# Autodesk Inventor assembly: COMPONENTS
(part 4 of 4)
- C:\Users\rtreacy\Documents\Inventor\SNAP Enclosure 8x10x1.75 Ver1.A\drawings\SNAP Ver2 pack-n-go\Workgroups\NotInProject\RESC3216X70N_R460.ipt
- C:\Users\rtreacy\Documents\Inventor\SNAP Enclosure 8x10x1.75 Ver1.A\drawings\SNAP Ver2 pack-n-go\Workgroups\NotInProject\RESC3216X70N_R165.ipt
- C:\Users\rtreacy\Documents\Inventor\SNAP Enclosure 8x10x1.75 Ver1.A\drawings\SNAP Ver2 pack-n-go\Workgroups\NotInProject\RESC3216X70N_R74.ipt
- C:\Users\rtreacy\Documents\Inventor\SNAP Enclosure 8x10x1.75 Ver1.A\drawings\SNAP Ver2 pack-n-go\Workgroups\NotInProject\RESC3216X70N_R474.ipt
- C:\Users\rtreacy\Documents\Inventor\SNAP Enclosure 8x10x1.75 Ver1.A\drawings\SNAP Ver2 pack-n-go\Workgroups\NotInProject\TP107_GNDTP6.ipt
- C:\Users\rtreacy\Documents\Inventor\SNAP Enclosure 8x10x1.75 Ver1.A\drawings\SNAP Ver2 pack-n-go\Workgroups\NotInProject\TP107_GNDTP5.ipt
- C:\Users\rtreacy\Documents\Inventor\SNAP Enclosure 8x10x1.75 Ver1.A\drawings\SNAP Ver2 pack-n-go\Workgroups\NotInProject\TP107_GNDTP4.ipt
- C:\Users\rtreacy\Documents\Inventor\SNAP Enclosure 8x10x1.75 Ver1.A\drawings\SNAP Ver2 pack-n-go\Workgroups\NotInProject\TP107_GNDTP3.ipt
- C:\Users\rtreacy\Documents\Inventor\SNAP Enclosure 8x10x1.75 Ver1.A\drawings\SNAP Ver2 pack-n-go\Workgroups\NotInProject\TP107_GNDTP2.ipt
- C:\Users\rtreacy\Documents\Inventor\SNAP Enclosure 8x10x1.75 Ver1.A\drawings\SNAP Ver2 pack-n-go\Workgroups\NotInProject\TP107_GNDTP1.ipt
- C:\Users\rtreacy\Documents\Inventor\SNAP Enclosure 8x10x1.75 Ver1.A\drawings\SNAP Ver2 pack-n-go\Workgroups\NotInProject\TP107_TP1.ipt
- C:\Users\rtreacy\Documents\Inventor\SNAP Enclosure 8x10x1.75 Ver1.A\drawings\SNAP Ver2 pack-n-go\Workgroups\NotInProject\TP107_TP4.ipt
- C:\Users\rtreacy\Documents\Inventor\SNAP Enclosure 8x10x1.75 Ver1.A\drawings\SNAP Ver2 pack-n-go\Workgroups\NotInProject\TP107_TP5.ipt
- C:\Users\rtreacy\Documents\Inventor\SNAP Enclosure 8x10x1.75 Ver1.A\drawings\SNAP Ver2 pack-n-go\Workgroups\NotInProject\TP107_TP10.ipt
- C:\Users\rtreacy\Documents\Inventor\SNAP Enclosure 8x10x1.75 Ver1.A\drawings\SNAP Ver2 pack-n-go\Workgroups\NotInProject\TP107_TP6.ipt
- C:\Users\rtreacy\Documents\Inventor\SNAP Enclosure 8x10x1.75 Ver1.A\drawings\SNAP Ver2 pack-n-go\Workgroups\NotInProject\TP107_TP8.ipt
- C:\Users\rtreacy\Documents\Inventor\SNAP Enclosure 8x10x1.75 Ver1.A\drawings\SNAP Ver2 pack-n-go\Workgroups\NotInProject\TP107_TP11.ipt
- C:\Users\rtreacy\Documents\Inventor\SNAP Enclosure 8x10x1.75 Ver1.A\drawings\SNAP Ver2 pack-n-go\Workgroups\NotInProject\TP107_TP7.ipt
- C:\Users\rtreacy\Documents\Inventor\SNAP Enclosure 8x10x1.75 Ver1.A\drawings\SNAP Ver2 pack-n-go\Workgroups\NotInProject\TP107_TP9.ipt
- C:\Users\rtreacy\Documents\Inventor\SNAP Enclosure 8x10x1.75 Ver1.A\drawings\SNAP Ver2 pack-n-go\Workgroups\NotInProject\DFN127P600X800X100-9T526X490N_U43.ipt
- C:\Users\rtreacy\Documents\Inventor\SNAP Enclosure 8x10x1.75 Ver1.A\drawings\SNAP Ver2 pack-n-go\Workgroups\NotInProject\SOP65P640X120-24L25N_U71.ipt
- C:\Users\rtreacy\Documents\Inventor\SNAP Enclosure 8x10x1.75 Ver1.A\drawings\SNAP Ver2 pack-n-go\Workgroups\NotInProject\TECONN_1734753-1_J10.ipt
## Components (800 placed, 793 different names)
1. INDC1005X55L_L30:1
2. INDC1005X55L_L31:1
3. NRAO-LOGO_NOREFDES:1
4. MOLEX_SD-74754-0220_M23:1
5. SHDRRA14W55P200_7X2_1665X100-1_J11:1
6. SHDRV14W55P200_7X2_1665X630H-1_J3:1
7. TE_CONN_6367550-5_P3:1
8. TO170P1430X470-6N-ALT1_U18:1
9. SMA_END_LAUNCH_SMATP1:1
10. SMA_END_LAUNCH_SMATP2:1
11. SMA_END_LAUNCH_SMATP3:1
12. SMA_END_LAUNCH_SMATP4:1
13. SMA_END_LAUNCH_SMATP5:1
14. SMA_END_LAUNCH_SMATP6:1
15. SMA_END_LAUNCH_SMATP7:1
16. SMA_END_LAUNCH_SMATP8:1
17. SMA_END_LAUNCH_SMATP9:1
18. SMA_END_LAUNCH_SMATP10:1
19. SMA_END_LAUNCH_SMATP11:1
20. SMA_END_LAUNCH_SMATP12:1
21. SMA_END_LAUNCH_SMATP13:1
22. SMA_END_LAUNCH_SMATP14:1
23. SMA_END_LAUNCH_SMATP15:1
24. SMA_END_LAUNCH_SMATP16:1
25. HDRV254W64P254R1L508T254H838_JP3:1
26. HDRV254W64P254R1L508T254H838_JP2:1
27. HDRV254W64P254R1L508T254H838_JP1:1
28. HDRV254W64P254R1L508T254H838_JP4:1
29. HDRV6X2_J9:1
30. HDRV6X2_J7:1
31. HDRV6X2_J5:1
32. HDRV6X2_J6:1
33. HDRV2X20_PI2:1
34. CAPPRD350W60D820H1170P_C259:1
35. CAPPRD350W60D820H1170P_C250:1
36. CAPPRD350W60D820H1170P_C241:1
37. CAPPRD350W60D820H1170P_C234:1
38. CAPPRD350W60D820H1170P_C227:1
39. QFN50P500X500X100-28N_U29:1
40. FID100X125_NOREFDES:1
41. FID100X125_NOREFDES:2
42. FID100X125_NOREFDES:3
43. FID100X125_NOREFDES:4
44. FID100X125_NOREFDES:5
45. FID100X125_NOREFDES:6
46. FID100X125_NOREFDES:7
47. FID100X125_NOREFDES:8
48. DIOAD1365W102L865D350B_D4:1
49. DIOAD1365W102L865D350B_D5:1
50. DIOAD1365W102L865D350B_D6:1
51. DIOAD1365W102L865D350B_D7:1
52. DIOAD1365W102L865D350B_D8:1
53. BGA676C100P26X26_2700X2700X260_U25:1
54. EMERSON_RFCONN_SMA-V_TP2:1
55. FIL_BNX01X_U24:1
56. MOLEX_744410010_P2:1
57. MOLEX_744410010_P1:1
58. SOT89_Q5:1
59. SOT89_Q6:1
60. QFN80P1000X1000X440-42T320X130X2N-ALT1_U20:1
61. HDR_1X2_LOCK_MOLEX_J61:1
62. DIOMELF3514_D14:1
63. SOT230P700X180-4L050N_Q17:1
64. QFP50P1400X1400X100-80N_U40:1
65. QFP50P1400X1400X100-80N_U42:1
66. QFN50P700X700X100-49T540X540L_U7:1
67. QFN50P700X700X100-49T540X540L_U2:1
68. QFN50P700X700X100-49T540X540L_U12:1
69. QFN50P500X500X100-33T320X320L_U21:1
70. QFN50P500X500X100-33T380X380L_U23:1
71. QFN50P400X400X100-25T280X280L_U22:1
72. DCDC-CONV_PTD08D210W-22N_U38:1
73. DCDC-CONV_PTD08D210W-22N_U36:1
74. DCDC-CONV_PTD08D210W-22N_U37:1
75. QFN50P300X300X100-17T178X178L_U17:1
76. QFN50P300X300X100-17T178X178L_U16:1
77. SOP65P640X120-16N_U41:1
78. SOP65P640X120-16N_U39:1
79. QFN40P260X180X55-16L_U28:1
80. QFN40P260X180X55-16L_U46:1
81. QFN40P260X180X55-16L_U47:1
82. DCDC-CONV_PTD08A020WAD-12N_U35:1
83. DCDC-CONV_PTD08A010WAD-12N_U34:1
84. HDRV1016W64P254R2L2032T905H900_J1:1
85. SW_SDA05H1SBD_S2:1
86. SW_SDA05H1SBD_S1:1
87. MOLEX_548190589_J4:1
88. SOP50P310X90-8N_U44:1
89. SOP50P310X90-8N_U45:1
90. OSC254P700X500X90-7T147X230N_U32:1
91. MOLEX_39301060_J2:1
92. SOT95P280X145-6N_U26:1
93. OSC254P700X500X90-6N_U48:1
94. OSC254P700X500X90-6N_U33:1
95. XFMR_TC1-1-13MG2_T11:1
96. XFMR_TC1-1-13MG2_T10:1
97. XFMR_TC1-1-13MG2_T4:1
98. XFMR_TC1-1-13MG2_T6:1
99. XFMR_TC1-1-13MG2_T12:1
100. XFMR_TC1-1-13MG2_T5:1
101. XFMR_TC1-1-13MG2_T3:1
102. XFMR_TC1-1-13MG2_T8:1
103. XFMR_TC1-1-13MG2_T9:1
104. XFMR_TC1-1-13MG2_T13:1
105. XFMR_TC1-1-13MG2_T2:1
106. XFMR_TC1-1-13MG2_T7:1
107. XFMR_TC1-1-13MG2_T1:1
108. SOT95P280X145-5N_U30:1
109. SOT95P280X145-5N_U19:1
110. SOT143R_X1:1
111. RESCAF65P100X100X45-4N_U10:1
112. RESCAF65P100X100X45-4N_U1:1
113. RESCAF65P100X100X45-4N_U11:1
114. RESCAF65P100X100X45-4N_U13:1
115. RESCAF65P100X100X45-4N_U14:1
116. RESCAF65P100X100X45-4N_U15:1
117. RESCAF65P100X100X45-4N_U3:1
118. RESCAF65P100X100X45-4N_U4:1
119. RESCAF65P100X100X45-4N_U5:1
120. RESCAF65P100X100X45-4N_U6:1
121. RESCAF65P100X100X45-4N_U8:1
122. RESCAF65P100X100X45-4N_U9:1
123. SW_TL3301EF100QG_SW5:1
124. SW_TL3301EF100QG_SW4:1
125. SW_TL3301EF100QG_SW3:1
126. SW_TL3301EF100QG_SW2:1
127. SW_TL3301EF100QG_SW1:1
128. SOT192P237X112-4L20N_D3:1
129. SOT95P237X100-4_Q1:1
130. SOT95P237X100-4_Q4:1
131. SOT95P237X100-4_Q3:1
132. SOT95P237X100-4_Q2:1
133. SOT95P237X100-4_Q8:1
134. SOT95P237X100-4_Q7:1
135. SOT95P240X110-3L16N_U31:1
136. SOT95P240X110-3L16N_D1:1
137. SOT95P240X110-3L16N_D2:1
138. CAPC1005X50L_C604:1
139. CAPC1005X50L_C603:1
140. CAPC1005X50L_C591:1
141. CAPC1005X50L_C592:1
142. CAPC1005X50L_C593:1
143. CAPC1005X50L_C46:1
144. CAPC1005X50L_C51:1
145. CAPC1005X50L_C57:1
146. CAPC1005X50L_C7:1
147. CAPC1005X50L_C82:1
148. CAPC1005X50L_C43:1
149. CAPC1005X50L_C96:1
150. CAPC1005X50L_C85:1
151. CAPC1005X50L_C90:1
152. CAPC1005X50L_C13:1
153. CAPC1005X50L_C4:1
154. CAPC1005X50L_C47:1
155. CAPC1005X50L_C5:1
156. CAPC1005X50L_C52:1
157. CAPC1005X50L_C58:1
158. CAPC1005X50L_C8:1
159. CAPC1005X50L_C83:1
160. CAPC1005X50L_C86:1
161. CAPC1005X50L_C91:1
162. CAPC1005X50L_C97:1
163. CAPC1005X50L_C19:1
164. CAPC1005X50L_C14:1
165. CAPC1005X50L_C17:1
166. CAPC1005X50L_C2:1
167. CAPC1005X50L_C41:1
168. CAPC1005X50L_C44:1
169. CAPC1005X50L_C53:1
170. CAPC1005X50L_C80:1
171. CAPC1005X50L_C87:1
172. CAPC1005X50L_C9:1
173. CAPC1005X50L_C92:1
174. CAPC1005X50L_C95:1
175. CAPC1005X50L_C48:1
176. CAPC1005X50L_C148:1
177. CAPC1005X50L_C56:1
178. CAPC1005X50L_C194:1
179. CAPC1005X50L_C195:1
180. CAPC1005X50L_C217:1
181. CAPC1005X50L_C219:1
182. CAPC1005X50L_C220:1
183. CAPC1005X50L_C222:1
184. CAPC1005X50L_C223:1
185. CAPC1005X50L_C224:1
186. CAPC1005X50L_C225:1
187. CAPC1005X50L_C226:1
188. CAPC1005X50L_C269:1
189. CAPC1005X50L_C270:1
190. CAPC1005X50L_C271:1
191. CAPC1005X50L_C273:1
192. CAPC1005X50L_C275:1
193. CAPC1005X50L_C276:1
194. CAPC1005X50L_C277:1
195. CAPC1005X50L_C285:1
196. CAPC1005X50L_C286:1
197. CAPC1005X50L_C291:1
198. CAPC1005X50L_C292:1
199. CAPC1005X50L_C293:1
200. CAPC1005X50L_C295:1
201. CAPC1005X50L_C297:1
202. CAPC1005X50L_C298:1
203. CAPC1005X50L_C299:1
204. CAPC1005X50L_C307:1
205. CAPC1005X50L_C308:1
206. CAPC1005X50L_C312:1
207. CAPC1005X50L_C313:1
208. CAPC1005X50L_C315:1
209. CAPC1005X50L_C317:1
210. CAPC1005X50L_C318:1
211. CAPC1005X50L_C319:1
212. CAPC1005X50L_C321:1
213. CAPC1005X50L_C323:1
214. CAPC1005X50L_C324:1
215. CAPC1005X50L_C325:1
216. CAPC1005X50L_C326:1
217. CAPC1005X50L_C327:1
218. CAPC1005X50L_C328:1
219. CAPC1005X50L_C15:1
220. CAPC1005X50L_C54:1
221. CAPC1005X50L_C192:1
222. CAPC1005X50L_C151:1
223. CAPC1005X50L_C152:1
224. CAPC1005X50L_C153:1
225. CAPC1005X50L_C154:1
226. CAPC1005X50L_C157:1
227. CAPC1005X50L_C160:1
228. CAPC1005X50L_C164:1
229. CAPC1005X50L_C167:1
230. CAPC1005X50L_C172:1
231. CAPC1005X50L_C176:1
232. CAPC1005X50L_C178:1
233. CAPC1005X50L_C16:1
234. CAPC1005X50L_C55:1
235. CAPC1005X50L_C94:1
236. CAPC1005X50L_C168:1
237. CAPC1005X50L_C173:1
238. CAPC1005X50L_C177:1
239. CAPC1005X50L_C180:1
240. CAPC1005X50L_C216:1
241. CAPC1005X50L_C184:1
242. CAPC1005X50L_C187:1
243. CAPC1005X50L_C188:1
244. CAPC1005X50L_C189:1
245. CAPC1005X50L_C182:1
246. CAPC1005X50L_C18:1
247. CAPC1005X50L_C93:1
248. CAPC1005X50L_C186:1
249. CAPC1005X50L_C20:1
250. CAPC1005X50L_C59:1
251. CAPC1005X50L_C98:1
252. CAPC1005X50L_C279:1
253. CAPC1005X50L_C280:1
254. CAPC1005X50L_C282:1
255. CAPC1005X50L_C284:1
256. CAPC1005X50L_C289:1
257. CAPC1005X50L_C301:1
258. CAPC1005X50L_C302:1
259. CAPC1005X50L_C304:1
260. CAPC1005X50L_C306:1
261. CAPC1005X50L_C311:1
262. CAPC1005X50L_C287:1
263. CAPC1005X50L_C309:1
264. CAPC1005X50L_C3:1
265. CAPC1005X50L_C42:1
266. CAPC1005X50L_C81:1
267. CAPC1005X50L_C45:1
268. CAPC1005X50L_C6:1
269. CAPC1005X50L_C84:1
270. CAPC1005X50L_C12:1
271. CAPC1005X50L_C181:1
272. CAPC1005X50L_C139:1
273. CAPC1005X50L_C76:1
274. CAPC1005X50L_C37:1
275. CAPC1005X50L_C115:1
276. CAPC1005X50L_C75:1
277. CAPC1005X50L_C36:1
278. CAPC1005X50L_C114:1
279. CAPC1005X50L_C74:1
280. CAPC1005X50L_C136:1
281. CAPC1005X50L_C183:1
282. CAPC1005X50L_C35:1
283. CAPC1005X50L_C113:1
284. CAPC1005X50L_C175:1
285. CAPC1005X50L_C174:1
286. CAPC1005X50L_C171:1
287. CAPC1005X50L_C166:1
288. CAPC1005X50L_C165:1
289. CAPC1005X50L_C185:1
290. CAPC1005X50L_C163:1
291. CAPC1005X50L_C72:1
292. CAPC1005X50L_C135:1
293. CAPC1005X50L_C131:1
294. CAPC1005X50L_C129:1
295. CAPC1005X50L_C127:1
296. CAPC1005X50L_C123:1
297. CAPC1005X50L_C33:1
298. CAPC1005X50L_C111:1
299. CAPC1005X50L_C89:1
300. CAPC1005X50L_C50:1
301. CAPC1005X50L_C11:1
302. CAPC1005X50L_C70:1
303. CAPC1005X50L_C31:1
304. CAPC1005X50L_C109:1
305. CAPC1005X50L_C69:1
306. CAPC1005X50L_C30:1
307. CAPC1005X50L_C121:1
308. CAPC1005X50L_C119:1
309. CAPC1005X50L_C108:1
310. CAPC1005X50L_C78:1
311. CAPC1005X50L_C39:1
312. CAPC1005X50L_C117:1
313. CAPC1005X50L_C104:1
314. CAPC1005X50L_C64:1
315. CAPC1005X50L_C1:1
316. CAPC1005X50L_C40:1
317. CAPC1005X50L_C79:1
318. CAPC1005X50L_C10:1
319. CAPC1005X50L_C49:1
320. CAPC1005X50L_C88:1
321. CAPC1005X50L_C67:1
322. CAPC1005X50L_C28:1
323. CAPC1005X50L_C106:1
324. CAPC1005X50L_C66:1
325. CAPC1005X50L_C27:1
326. CAPC1005X50L_C105:1
327. CAPC1005X50L_C65:1
328. CAPC1005X50L_C26:1
329. CAPC1005X50L_C25:1
330. CAPC1005X50L_C102:1
331. CAPC1005X50L_C103:1
332. CAPC1005X50L_C63:1
333. CAPC1005X50L_C24:1
334. CAPC1005X50L_C61:1
335. CAPC1005X50L_C100:1
336. CAPC1005X50L_C22:1
337. CAPC1005X50L_C601:1
338. CAPC1005X50L_C602:1
339. CAPC1608X90N_C120:1
340. CAPC1608X90N_C124:1
341. CAPC1608X90N_C128:1
342. CAPC1608X90N_C132:1
343. CAPC1608X90N_C179:1
344. CAPC1608X90N_C150:1
345. CAPC1608X90N_C140:1
346. CAPC1608X90N_C161:1
347. CAPC1608X90N_C169:1
348. CAPC1608X90N_C190:1
349. CAPC1608X90N_C218:1
350. CAPC1608X90N_C221:1
351. CAPC1608X90N_C229:1
352. CAPC1608X90N_C236:1
353. CAPC1608X90N_C243:1
354. CAPC1608X90N_C252:1
355. CAPC1608X90N_C261:1
356. CAPC1608X90N_C193:1
357. CAPC1608X90N_C215:1
358. CAPC1608X90N_C21:1
359. CAPC1608X90N_C60:1
360. CAPC1608X90N_C99:1
361. CAPC1608X90N_C38:1
362. CAPC1608X90N_C116:1
363. CAPC1608X90N_C73:1
364. CAPC1608X90N_C34:1
365. CAPC1608X90N_C112:1
366. CAPC1608X90N_C71:1
367. CAPC1608X90N_C32:1
368. CAPC1608X90N_C110:1
369. CAPC1608X90N_C77:1
370. CAPC1608X90N_C68:1
371. CAPC1608X90N_C29:1
372. CAPC1608X90N_C107:1
373. CAPC1608X90N_C62:1
374. CAPC1608X90N_C23:1
375. CAPC1608X90N_C101:1
376. CAPC3216X180N_C134:1
377. CAPC3216X180N_C138:1
378. CAPC3216X180N_C141:1
379. CAPC3216X180N_C143:1
380. CAPC3216X180N_C144:1
381. CAPC3216X180N_C231:1
382. CAPC3216X180N_C238:1
383. CAPC3216X180N_C245:1
384. CAPC3216X180N_C254:1
385. CAPC3216X180N_C263:1
386. CAPC3216X180N_C314:1
387. CAPC3216X180N_C316:1
388. CAPC3216X180N_C320:1
389. CAPC3216X180N_C322:1
390. CAPC3216X180N_C146:1
391. CAPC3216X180N_C197:1
392. CAPC3216X180N_C145:1
393. CAPC3216X180N_C149:1
394. CAPC3216X180N_C155:1
395. CAPC3216X180N_C158:1
396. CAPC3216X180N_C156:1
397. CAPC3216X180N_C159:1
398. CAPC3216X180N_C212:1
399. CAPC3216X180N_C213:1
400. CAPC3216X180N_C214:1
401. CAPC3216X180N_C228:1
402. CAPC3216X180N_C235:1
403. CAPC3216X180N_C242:1
404. CAPC3216X180N_C251:1
405. CAPC3216X180N_C260:1
406. CAPC3216X180N_C232:1
407. CAPC3216X180N_C239:1
408. CAPC3216X180N_C246:1
409. CAPC3216X180N_C255:1
410. CAPC3216X180N_C264:1
411. CAPC3216X180N_C248:1
412. CAPC3216X180N_C257:1
413. CAPC3216X180N_C266:1
414. CAPC3216X180N_C268:1
415. CAPC3216X180N_C290:1
416. CAPMP7343X310N-ALT1_C137:1
417. CAPMP7343X310N-ALT1_C233:1
418. CAPMP7343X310N-ALT1_C240:1
419. CAPMP7343X310N-ALT1_C247:1
420. CAPMP7343X310N-ALT1_C249:1
421. CAPMP7343X310N-ALT1_C256:1
422. CAPMP7343X310N-ALT1_C258:1
423. CAPMP7343X310N-ALT1_C265:1
424. CAPMP7343X310N-ALT1_C267:1
425. CAPC3225X270N_C414:1
426. CAPC3225X270N_C142:1
427. CAPC3225X270N_C147:1
428. CAPC3225X270N_C198:1
429. CAPC3225X270N_C199:1
430. CAPC3225X270N_C200:1
431. CAPC3225X270N_C201:1
432. CAPC3225X270N_C202:1
433. CAPC3225X270N_C203:1
434. CAPC3225X270N_C204:1
435. CAPC3225X270N_C205:1
436. CAPC3225X270N_C208:1
437. CAPC2012X105N_C162:1
438. CAPC1005X50N_C170:1
439. CAPAE830X1050D995DD305L335N_C191:1
440. CAPAE830X1050D995DD305L335N_C230:1
441. CAPAE830X1050D995DD305L335N_C237:1
442. CAPAE830X1050D995DD305L335N_C244:1
443. CAPAE830X1050D995DD305L335N_C253:1
444. CAPAE830X1050D995DD305L335N_C262:1
445. CAPMP7343X180N-ALT1_C402:1
446. CAPMP7343X180N-ALT1_C413:1
447. CAPMP7343X180N-ALT1_C400:1
448. CAPMP7343X180N-ALT1_C401:1
449. CAPMP7343X180N-ALT1_C206:1
450. CAPMP7343X180N-ALT1_C207:1
451. CAPC2012X140N_C419:1
452. CAPC2012X140N_C420:1
453. CAPC2012X140N_C410:1
454. CAPC2012X140N_C418:1
455. CAPC2012X140N_C417:1
456. CAPC2012X140N_C416:1
457. CAPC2012X140N_C415:1
458. CAPC2012X140N_C412:1
459. CAPC2012X140N_C411:1
460. CAPC2012X140N_C408:1
461. CAPC2012X140N_C409:1
462. CAPC2012X140N_C404:1
463. CAPC2012X140N_C407:1
464. CAPC2012X140N_C406:1
465. CAPC2012X140N_C405:1
466. CAPC2012X140N_C403:1
467. CAPC2012X140N_C209:1
468. CAPC2012X140N_C210:1
469. CAPC2012X140N_C211:1
470. CAPC2012X140N_C272:1
471. CAPC2012X140N_C274:1
472. CAPC2012X140N_C294:1
473. CAPC2012X140N_C296:1
474. CAPC2012X140N_C133:1
475. CAPC2012X140N_C130:1
476. CAPC2012X140N_C126:1
477. CAPC2012X140N_C125:1
478. CAPC2012X140N_C122:1
479. CAPC2012X140N_C118:1
480. CAPC0603X30L_C278:1
481. CAPC0603X30L_C281:1
482. CAPC0603X30L_C283:1
483. CAPC0603X30L_C288:1
484. CAPC0603X30L_C300:1
485. CAPC0603X30L_C303:1
486. CAPC0603X30L_C305:1
487. CAPC0603X30L_C310:1
488. SOD3717X135_D10:1
489. SOD3717X135_D9:1
490. LEDM180X60X60N_DS1:1
491. LEDM180X60X60N_DS10:1
492. LEDM180X60X60N_DS11:1
493. LEDM180X60X60N_DS4:1
494. LEDM180X60X60N_DS5:1
495. LEDM180X60X60N_DS7:1
496. LEDM180X60X60N_DS8:1
497. LEDM180X60X60N_DS9:1
498. LEDM180X60X60N_DS2:1
499. LEDM180X60X60N_DS3:1
500. INDM4532X340N_L1:1
501. INDM4532X340N_L10:1
502. INDM4532X340N_L11:1
503. INDM4532X340N_L12:1
504. INDM4532X340N_L2:1
505. INDM4532X340N_L3:1
506. INDM4532X340N_L4:1
507. INDM4532X340N_L5:1
508. INDM4532X340N_L6:1
509. INDM4532X340N_L8:1
510. INDM4532X340N_L7:1
511. INDM4532X340N_L9:1
512. INDC2012X110N_L14:1
513. INDC2012X110N_L13:1
514. INDM9630X305N_L15:1
515. INDM9630X305N_L16:1
516. INDM9630X305N_L17:1
517. INDM9630X305N_L18:1
518. INDM9630X305N_L19:1
519. INDC1608X95L-ALT1_L20:1
520. INDC1608X95L-ALT1_L21:1
521. INDC1608X95L-ALT1_L23:1
522. INDC1608X95L-ALT1_L22:1
523. INDM5551X200N_L24:1
524. INDM5551X200N_L25:1
525. INDM5551X200N_L26:1
526. INDM5551X200N_L27:1
527. RESC1005X35N_R443:1
528. RESC1005X35N_R442:1
529. RESC1005X35N_R438:1
530. RESC1005X35N_R437:1
531. RESC1005X35N_R436:1
532. RESC1005X35N_R434:1
533. RESC1005X35N_R114:1
534. RESC1005X35N_R133:1
535. RESC1005X35N_R135:1
536. RESC1005X35N_R139:1
537. RESC1005X35N_R432:1
538. RESC1005X35N_R431:1
539. RESC1005X35N_R427:1
540. RESC1005X35N_R426:1
541. RESC1005X35N_R424:1
542. RESC1005X35N_R423:1
543. RESC1005X35N_R421:1
544. RESC1005X35N_R420:1
545. RESC1005X35N_R433:1
546. RESC1005X35N_R428:1
547. RESC1005X35N_R425:1
548. RESC1005X35N_R422:1
549. RESC1005X35N_R1:1
550. RESC1005X35N_R12:1
551. RESC1005X35N_R13:1
552. RESC1005X35N_R16:1
553. RESC1005X35N_R21:1
554. RESC1005X35N_R25:1
555. RESC1005X35N_R26:1
556. RESC1005X35N_R28:1
557. RESC1005X35N_R29:1
558. RESC1005X35N_R32:1
559. RESC1005X35N_R33:1
560. RESC1005X35N_R36:1
561. RESC1005X35N_R41:1
562. RESC1005X35N_R45:1
563. RESC1005X35N_R46:1
564. RESC1005X35N_R48:1
565. RESC1005X35N_R49:1
566. RESC1005X35N_R5:1
567. RESC1005X35N_R52:1
568. RESC1005X35N_R53:1
569. RESC1005X35N_R56:1
570. RESC1005X35N_R6:1
571. RESC1005X35N_R8:1
572. RESC1005X35N_R9:1
573. RESC1005X35N_R10:1
574. RESC1005X35N_R14:1
575. RESC1005X35N_R2:1
576. RESC1005X35N_R22:1
577. RESC1005X35N_R24:1
578. RESC1005X35N_R30:1
579. RESC1005X35N_R34:1
580. RESC1005X35N_R4:1
581. RESC1005X35N_R42:1
582. RESC1005X35N_R44:1
583. RESC1005X35N_R50:1
584. RESC1005X35N_R54:1
585. RESC1005X35N_R100:1
586. RESC1005X35N_R102:1
587. RESC1005X35N_R103:1
588. RESC1005X35N_R104:1
589. RESC1005X35N_R105:1
590. RESC1005X35N_R106:1
591. RESC1005X35N_R96:1
592. RESC1005X35N_R97:1
593. RESC1005X35N_R109:1
594. RESC1005X35N_R140:1
595. RESC1005X35N_R145:1
596. RESC1005X35N_R146:1
597. RESC1005X35N_R147:1
598. RESC1005X35N_R148:1
599. RESC1005X35N_R154:1
600. RESC1005X35N_R157:1
601. RESC1005X35N_R158:1
602. RESC1005X35N_R159:1
603. RESC1005X35N_R160:1
604. RESC1005X35N_R161:1
605. RESC1005X35N_R162:1
606. RESC1005X35N_R163:1
607. RESC1005X35N_R164:1
608. RESC1005X35N_R194:1
609. RESC1005X35N_R195:1
610. RESC1005X35N_R196:1
611. RESC1005X35N_R201:1
612. RESC1005X35N_R202:1
613. RESC1005X35N_R203:1
614. RESC1005X35N_R204:1
615. RESC1005X35N_R205:1
616. RESC1005X35N_R206:1
617. RESC1005X35N_R207:1
618. RESC1005X35N_R208:1
619. RESC1005X35N_R210:1
620. RESC1005X35N_R211:1
621. RESC1005X35N_R212:1
622. RESC1005X35N_R213:1
623. RESC1005X35N_R214:1
624. RESC1005X35N_R215:1
625. RESC1005X35N_R216:1
626. RESC1005X35N_R217:1
627. RESC1005X35N_R218:1
628. RESC1005X35N_R219:1
629. RESC1005X35N_R221:1
630. RESC1005X35N_R222:1
631. RESC1005X35N_R223:1
632. RESC1005X35N_R224:1
633. RESC1005X35N_R226:1
634. RESC1005X35N_R227:1
635. RESC1005X35N_R11:1
636. RESC1005X35N_R15:1
637. RESC1005X35N_R23:1
638. RESC1005X35N_R27:1
639. RESC1005X35N_R3:1
640. RESC1005X35N_R31:1
641. RESC1005X35N_R35:1
642. RESC1005X35N_R43:1
643. RESC1005X35N_R47:1
644. RESC1005X35N_R51:1
645. RESC1005X35N_R55:1
646. RESC1005X35N_R7:1
647. RESC1005X35N_R110:1
648. RESC1005X35N_R112:1
649. RESC1005X35N_R113:1
650. RESC1005X35N_R115:1
651. RESC1005X35N_R116:1
652. RESC1005X35N_R120:1
653. RESC1005X35N_R124:1
654. RESC1005X35N_R111:1
655. RESC1005X35N_R117:1
656. RESC1005X35N_R119:1
657. RESC1005X35N_R123:1
658. RESC1005X35N_R130:1
659. RESC1005X35N_R132:1
660. RESC1005X35N_R134:1
661. RESC1005X35N_R137:1
662. RESC1005X35N_R170:1
663. RESC1005X35N_R171:1
664. RESC1005X35N_R175:1
665. RESC1005X35N_R178:1
666. RESC1005X35N_R183:1
667. RESC1005X35N_R184:1
668. RESC1005X35N_R188:1
669. RESC1005X35N_R191:1
670. RESC1005X35N_R118:1
671. RESC1005X35N_R121:1
672. RESC1005X35N_R126:1
673. RESC1005X35N_R131:1
674. RESC1005X35N_R122:1
675. RESC1005X35N_R125:1
676. RESC1005X35N_R138:1
677. RESC1005X35N_R127:1
678. RESC1005X35N_R128:1
679. RESC1005X35N_R166:1
680. RESC1005X35N_R167:1
681. RESC1005X35N_R169:1
682. RESC1005X35N_R172:1
683. RESC1005X35N_R173:1
684. RESC1005X35N_R174:1
685. RESC1005X35N_R176:1
686. RESC1005X35N_R177:1
687. RESC1005X35N_R179:1
688. RESC1005X35N_R180:1
689. RESC1005X35N_R182:1
690. RESC1005X35N_R185:1
691. RESC1005X35N_R186:1
692. RESC1005X35N_R187:1
693. RESC1005X35N_R189:1
694. RESC1005X35N_R190:1
695. RESC1005X35N_R136:1
696. RESC1005X35N_R141:1
697. RESC1005X35N_R142:1
698. RESC1005X35N_R143:1
699. RESC1005X35N_R144:1
700. RESC1005X35N_R197:1
701. RESC1005X35N_R198:1
702. RESC1005X35N_R199:1
703. RESC1005X35N_R200:1
704. RESC1005X35N_R155:1
705. RESC1005X35N_R156:1
706. RESC1005X35N_R225:1
707. RESC1005X35N_R228:1
708. RESC1005X35N_R229:1
709. RESC1005X35N_R230:1
710. RESC1005X35N_R231:1
711. RESC1005X35N_R232:1
712. RESC1005X35N_R233:1
713. RESC1005X35N_R234:1
714. RESC1005X35N_R168:1
715. RESC1005X35N_R181:1
716. RESC1005X35N_R17:1
717. RESC1005X35N_R18:1
718. RESC1005X35N_R37:1
719. RESC1005X35N_R38:1
720. RESC1005X35N_R57:1
721. RESC1005X35N_R58:1
722. RESC1005X35N_R19:1
723. RESC1005X35N_R39:1
724. RESC1005X35N_R59:1
725. RESC1005X35N_R20:1
726. RESC1005X35N_R40:1
727. RESC1005X35N_R60:1
728. RESC1005X35N_R209:1
729. RESC1005X35N_R220:1
730. RESC1005X35N_R61:1
731. RESC1005X35N_R65:1
732. RESC1005X35N_R67:1
733. RESC1005X35N_R62:1
734. RESC1005X35N_R64:1
735. RESC1005X35N_R63:1
736. RESC1005X35N_R66:1
737. RESC1005X35N_R70:1
738. RESC1005X35N_R71:1
739. RESC1005X35N_R72:1
740. RESC1005X35N_R73:1
741. RESC1005X35N_R75:1
742. RESC1005X35N_R76:1
743. RESC1005X35N_R77:1
744. RESC1005X35N_R91:1
745. RESC1005X35N_R92:1
746. RESC1005X35N_R94:1
747. RESC1005X35N_R95:1
748. RESC1005X35N_R80:1
749. RESC1005X35N_R81:1
750. RESC1005X35N_R82:1
751. RESC1005X35N_R83:1
752. RESC1005X35N_R84:1
753. RESC1005X35N_R86:1
754. RESC1005X35N_R90:1
755. RESC1005X35N_R93:1
756. RESC1005X35N_R99:1
757. RESC1005X35N_R85:1
758. RESC1005X35N_R87:1
759. RESC1005X35N_R407:1
760. RESC1005X35N_R408:1
761. RESC1608X50N_R441:1
762. RESC1608X50N_R440:1
763. RESC1608X50N_R439:1
764. RESC1608X50N_R435:1
765. RESC1608X50N_R101:1
766. RESC1608X50N_R107:1
767. RESC1608X50N_R108:1
768. RESC1608X50N_R78:1
769. RESC1608X50N_R79:1
770. RESC1608X50N_R88:1
771. RESC1608X50N_R89:1
772. RESC1608X50N_R98:1
773. RESC1608X50N_R192:1
774. RESC1608X50N_R193:1
775. RESC1608X50N_R149:1
776. RESC1608X50N_R153:1
777. RESC1608X50N_R68:1
778. RESC1608X50N_R69:1
779. RESC3216X70N_R460:1
780. RESC3216X70N_R165:1
781. RESC3216X70N_R74:1
782. RESC3216X70N_R474:1
783. TP107_GNDTP6:1
784. TP107_GNDTP5:1
785. TP107_GNDTP4:1
786. TP107_GNDTP3:1
787. TP107_GNDTP2:1
788. TP107_GNDTP1:1
789. TP107_TP1:1
790. TP107_TP4:1
791. TP107_TP5:1
792. TP107_TP10:1
793. TP107_TP6:1
794. TP107_TP8:1
795. TP107_TP11:1
796. TP107_TP7:1
797. TP107_TP9:1
798. DFN127P600X800X100-9T526X490N_U43:1
799. SOP65P640X120-24L25N_U71:1
800. TECONN_1734753-1_J10:1
